# Autodesk Inventor assembly: 装配体
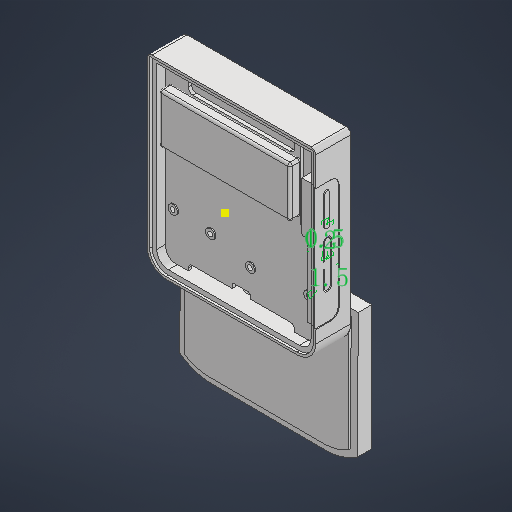
[picture p0: Inventor's stored thumbnail of the model, 512x512]
Saved by Autodesk Inventor 2025 (Build 290162000, 162)
## iProperties
Created: 2025-10-27
Part Number: 装配体
Document SubType Name: Assembly
Designer: XH
Author: XH
## Documents named in this file (9)
- D:\三星\装配体.iam
- D:\三星\键盘外壳.ipt
- D:\三星\电子\摄像头电路部分.ipt
- D:\三星\电子\上板电池.ipt
- D:\三星\电子\屏幕.ipt
- D:\三星\第二层板.ipt
- D:\三星\电子\大电池包裹.ipt
- D:\三星\dlc.iam
- D:\三星\部件1.iam
## Components (8 placed, 8 different names)
1. 键盘外壳:1 — 配合:16, 配合:17, 配合:21, 配合:22, 配合:23
2. 摄像头电路部分:1 — 配合:10, 配合:13, 表面齐平:3
3. 上板电池:1 — 配合:20, 表面齐平:3
4. 屏幕:1 — 配合:10
5. 第二层板:1 — 配合:13, 配合:20
6. 大电池包裹:1 — 配合:16, 配合:17
7. dlc:1 [sub-assembly] — 配合:21, 配合:22
8. 部件1:1 [sub-assembly] — 配合:23
## Relationships (9: Mate 8, Flush 1)
- 配合:20 [Mate]: 上板电池:1 ↔ 第二层板:1
- 配合:10 [Mate] (0.1 mm): 摄像头电路部分:1 ↔ 屏幕:1
- 配合:13 [Mate]: 摄像头电路部分:1 ↔ 第二层板:1
- 配合:16 [Mate]: 键盘外壳:1 ↔ 大电池包裹:1
- 配合:17 [Mate]: 键盘外壳:1 ↔ 大电池包裹:1
- 表面齐平:3 [Flush] (-6 mm): 摄像头电路部分:1 ↔ 上板电池:1
- 配合:21 [Mate]: 键盘外壳:1 ↔ dlc:1
- 配合:22 [Mate]: 键盘外壳:1 ↔ dlc:1
- 配合:23 [Mate]: 键盘外壳:1 ↔ 部件1:1
